# Autodesk Inventor assembly: Bumper Assemby
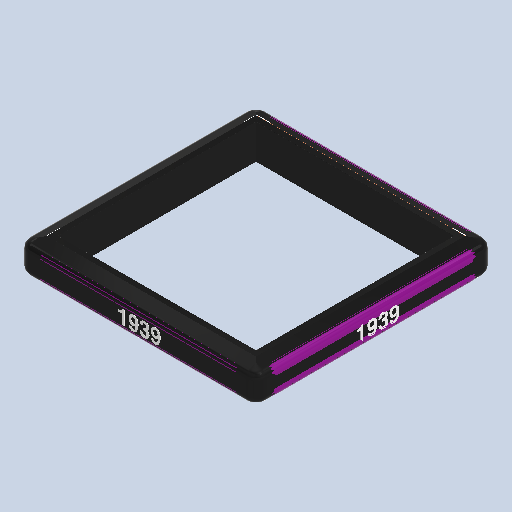
[picture p0: Inventor's stored thumbnail of the model, 512x512]
Saved by Autodesk Inventor 2023.3 (Build 273359000, 359)
## iProperties
Created: 2023-11-22
Part Number: Bumper Assemby
Document SubType Name: Assembly
Designer: adamarnold
Author: adamarnold
## Documents named in this file (6)
- D:\.shortcut-targets-by-id\104lhnwPhYvankLacu8RGROV89Bx_24Mg\1939\2_Design\2023-2024\Parts\Bumpers\Bumper Assemby.iam
- D:\.shortcut-targets-by-id\104lhnwPhYvankLacu8RGROV89Bx_24Mg\1939\2_Design\2023-2024\Parts\Bumpers\Bumper wood.ipt
- D:\.shortcut-targets-by-id\104lhnwPhYvankLacu8RGROV89Bx_24Mg\1939\2_Design\2023-2024\Parts\Cut Stock\2x2 Angle\2” x 2” x 0.090” bumper corner.ipt
- D:\.shortcut-targets-by-id\104lhnwPhYvankLacu8RGROV89Bx_24Mg\1939\2_Design\2023-2024\Parts\Bumpers\Pool Noodles.ipt
- D:\.shortcut-targets-by-id\104lhnwPhYvankLacu8RGROV89Bx_24Mg\1939\2_Design\2023-2024\Parts\Bumpers\Cover.ipt
- D:\.shortcut-targets-by-id\104lhnwPhYvankLacu8RGROV89Bx_24Mg\1939\2_Design\2023-2024\Parts\Bumpers\Numbers.ipt
## Components (15 placed, 6 different names)
1. First Piece Locked Down — Flush:1, Flush:2, Mate:1, Flush:3, Flush:4, Flush:5, Flush:9, Mate:6, Mate:8, Flush:15
2. Bumper wood:1 — Flush:3, Flush:4, Flush:5, Flush:6, Flush:7, Flush:8, Mate:3, Mate:9, Flush:17
3. Bumper wood:3 — Flush:6, Flush:7, Flush:8, Flush:10, Flush:11, Mate:2, Flush:12, Mate:5, Flush:16, Mate:10, Flush:22
4. Bumper wood:4 — Flush:9, Flush:10, Flush:11, Mate:4, Flush:13, Mate:7, Flush:14, Flush:21, Flush:23
5. 2” x 2” x 0.090” bumper corner:1 — Mate:2, Mate:3, Flush:12
6. 2” x 2” x 0.090” bumper corner:2 — Mate:4, Mate:5, Flush:13
7. 2” x 2” x 0.090” bumper corner:3 — Mate:6, Mate:7, Flush:14
8. 2” x 2” x 0.090” bumper corner:4 — Mate:8, Mate:9, Flush:15
9. Pool Noodles:1 — Flush:16, Flush:17, Mate:10, Flush:18, Flush:19, Flush:20
10. Pool Noodles:2 — Flush:18, Flush:19, Flush:20
11. Cover:1 — Flush:21, Flush:22, Flush:23, Mate:11, Flush:24, Flush:25, Mate:12, Flush:26, Flush:27, Mate:13, Flush:28, Flush:29, Mate:14, Flush:30, Flush:31
12. Numbers:1 — Mate:11, Flush:24, Flush:25
13. Numbers:2 — Mate:12, Flush:26, Flush:27
14. Numbers:3 — Mate:13, Flush:28, Flush:29
15. Numbers:4 — Mate:14, Flush:30, Flush:31
## Relationships (45: Flush 31, Mate 14)
- Flush:1: First Piece Locked Down
- Flush:2: First Piece Locked Down
- Mate:1: First Piece Locked Down
- Flush:3: First Piece Locked Down ↔ Bumper wood:1
- Flush:4: First Piece Locked Down ↔ Bumper wood:1
- Flush:5: First Piece Locked Down ↔ Bumper wood:1
- Flush:6: Bumper wood:1 ↔ Bumper wood:3
- Flush:7: Bumper wood:1 ↔ Bumper wood:3
- Flush:8: Bumper wood:1 ↔ Bumper wood:3
- Flush:9: First Piece Locked Down ↔ Bumper wood:4
- Flush:10: Bumper wood:3 ↔ Bumper wood:4
- Flush:11: Bumper wood:3 ↔ Bumper wood:4
- Mate:2: Bumper wood:3 ↔ 2” x 2” x 0.090” bumper corner:1
- Mate:3: Bumper wood:1 ↔ 2” x 2” x 0.090” bumper corner:1
- Flush:12: Bumper wood:3 ↔ 2” x 2” x 0.090” bumper corner:1
- Mate:4: Bumper wood:4 ↔ 2” x 2” x 0.090” bumper corner:2
- Mate:5: Bumper wood:3 ↔ 2” x 2” x 0.090” bumper corner:2
- Flush:13: Bumper wood:4 ↔ 2” x 2” x 0.090” bumper corner:2
- Mate:6: First Piece Locked Down ↔ 2” x 2” x 0.090” bumper corner:3
- Mate:7: Bumper wood:4 ↔ 2” x 2” x 0.090” bumper corner:3
- Flush:14: Bumper wood:4 ↔ 2” x 2” x 0.090” bumper corner:3
- Mate:8: First Piece Locked Down ↔ 2” x 2” x 0.090” bumper corner:4
- Mate:9: Bumper wood:1 ↔ 2” x 2” x 0.090” bumper corner:4
- Flush:15: First Piece Locked Down ↔ 2” x 2” x 0.090” bumper corner:4
- Flush:16 (-25.4 mm): Bumper wood:3 ↔ Pool Noodles:1
- Flush:17 (-25.4 mm): Bumper wood:1 ↔ Pool Noodles:1
- Mate:10 (-34.925 mm): Bumper wood:3 ↔ Pool Noodles:1
- Flush:18: Pool Noodles:1 ↔ Pool Noodles:2
- Flush:19 (-50.8 mm): Pool Noodles:1 ↔ Pool Noodles:2
- Flush:20: Pool Noodles:1 ↔ Pool Noodles:2
- Flush:21 (-0.635 mm): Bumper wood:4 ↔ Cover:1
- Flush:22 (-0.635 mm): Bumper wood:3 ↔ Cover:1
- Flush:23 (-0.635 mm): Bumper wood:4 ↔ Cover:1
- Mate:11: Cover:1 ↔ Numbers:1
- Flush:24 (35.56 mm): Cover:1 ↔ Numbers:1
- Flush:25 (349.25 mm): Cover:1 ↔ Numbers:1
- Mate:12: Cover:1 ↔ Numbers:2
- Flush:26 (35.56 mm): Cover:1 ↔ Numbers:2
- Flush:27 (349.25 mm): Cover:1 ↔ Numbers:2
- Mate:13: Cover:1 ↔ Numbers:3
- Flush:28 (35.56 mm): Cover:1 ↔ Numbers:3
- Flush:29 (349.25 mm): Cover:1 ↔ Numbers:3
- Mate:14: Cover:1 ↔ Numbers:4
- Flush:30 (349.25 mm): Cover:1 ↔ Numbers:4
- Flush:31 (35.56 mm): Cover:1 ↔ Numbers:4
